# Autodesk Inventor assembly: カート
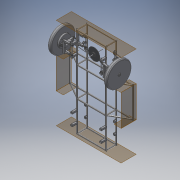
[picture p0: Inventor's stored thumbnail of the model, 180x180]
Saved by Autodesk Inventor 2018 (Build 220112000, 112)
## iProperties
Created: 2017-10-07
Part Number: カート
Material: 一般
Document SubType Name: Assembly
Designer: Kosei
Author: Kosei
## Documents named in this file (17)
- C:\Users\mura5\Documents\RBBR\CAD\カート.iam
- C:\Users\mura5\Documents\RBBR\CAD\シャーシ\シャーシ.iam
- C:\Users\mura5\Documents\RBBR\CAD\サスペンション\上アーム(前).iam
- C:\Users\mura5\Documents\RBBR\CAD\汎用部品\シャフト12x300mm.ipt
- C:\Users\mura5\Documents\RBBR\CAD\サスペンション\下アーム(前後).iam
- C:\Users\mura5\Documents\RBBR\CAD\サスペンション\車軸受け(前,左).iam
- C:\Users\mura5\Documents\RBBR\CAD\汎用部品\シャフト10x230mm.ipt
- C:\Users\mura5\Documents\RBBR\CAD\サスペンション\スプリング\スプリング.iam
- C:\Users\mura5\Documents\RBBR\CAD\車輪\前輪.ipt
- C:\Users\mura5\Documents\RBBR\CAD\車輪\前輪シャフト.ipt
- C:\Users\mura5\Documents\RBBR\CAD\車輪\前輪シャフトワッシャー.ipt
- C:\Users\mura5\Documents\RBBR\CAD\サスペンション\車軸受け(前,右).iam
- C:\Users\mura5\Documents\RBBR\CAD\ステアリング\ロッド.iam
- C:\Users\mura5\Documents\RBBR\CAD\ステアリング\車輪側スプロケット.ipt
- C:\Users\mura5\Documents\RBBR\CAD\装飾(仮)\前後.ipt
- C:\Users\mura5\Documents\RBBR\CAD\装飾(仮)\左右.ipt
- C:\Users\mura5\Documents\RBBR\CAD\装飾(仮)\泥除け1.ipt
## Components (33 placed, 16 different names)
1. シャーシ:1 [sub-assembly] — フラッシュ:2, フラッシュ:3, フラッシュ:4, 円柱状:1, フラッシュ:5, 円柱状:2, フラッシュ:6, 円柱状:3, フラッシュ:7, 円柱状:4, フラッシュ:8, メイト:1, メイト:2, メイト:3, メイト:4, フラッシュ:9, フラッシュ:10, メイト:5, フラッシュ:11, メイト:6, フラッシュ:12, 角度:3, メイト:7, フラッシュ:13, フラッシュ:14, メイト:8, フラッシュ:15, フラッシュ:16, メイト:9, フラッシュ:17, フラッシュ:18, メイト:10, フラッシュ:19, メイト:11, メイト:12, フラッシュ:25, メイト:15, メイト:17
2. 泥除け1:1 — メイト:11, フラッシュ:24, メイト:13
3. 泥除け1:2 — メイト:15, フラッシュ:26, メイト:16
4. 泥除け1:3 — メイト:12, フラッシュ:23, メイト:14
5. 泥除け1:4 — メイト:17, フラッシュ:27, メイト:18
6. シャフト12x300mm:1 — 円柱状:1, フラッシュ:5, 円柱状:5, 円柱状:11
7. シャフト12x300mm:3 — 円柱状:3, フラッシュ:7, 円柱状:7
8. シャフト10x230mm:1 — 円柱状:9, フラッシュ:9, 円柱状:12
9. 上アーム(前):1 [sub-assembly] — 円柱状:5, メイト:1, リジッド:1, 角度:4
10. 下アーム(前後):1 [sub-assembly] — 円柱状:7, メイト:3, リジッド:2, 円柱状:9
11. 車軸受け(前,左):1 [sub-assembly] — リジッド:1, リジッド:2, 回転:2, リジッド:9
12. スプリング:1 [sub-assembly] — 円柱状:11, 円柱状:12
13. 前輪:1 — 回転:1, リジッド:5, 角度:8
14. 前輪シャフト:1 — 回転:1
15. 前輪シャフトワッシャー:1 — リジッド:5, 回転:2
16. シャフト12x300mm:2 — 円柱状:2, フラッシュ:6, 円柱状:6, 円柱状:13
17. シャフト12x300mm:4 — 円柱状:4, フラッシュ:8, 円柱状:8
18. シャフト10x230mm:2 — フラッシュ:10, 円柱状:10, 円柱状:14
19. 上アーム(前):2 [sub-assembly] — 円柱状:6, メイト:2, リジッド:3, 角度:5
20. 下アーム(前後):2 [sub-assembly] — 円柱状:8, メイト:4, リジッド:4, 円柱状:10
21. 車軸受け(前,右):1 [sub-assembly] — リジッド:3, リジッド:4, 回転:3, リジッド:8
22. スプリング:2 [sub-assembly] — 円柱状:13, 円柱状:14
23. 前輪:2 — リジッド:6, リジッド:7
24. 前輪シャフト:2 — リジッド:6
25. 前輪シャフトワッシャー:2 — リジッド:7, 回転:3
26. ロッド:1 [sub-assembly] — リジッド:8, リジッド:12, 角度:6
27. ロッド:2 [sub-assembly] — リジッド:9, リジッド:13, 角度:7
28. 車輪側スプロケット:1 — 円柱状:15, フラッシュ:12, リジッド:12, リジッド:13, 角度:3, 角度:6, 角度:7
29. シャフト12x300mm:5 — メイト:5, フラッシュ:11, メイト:6, 円柱状:15
30. 前後:1 — メイト:7, フラッシュ:13, フラッシュ:14
31. 前後:2 — メイト:8, フラッシュ:15, フラッシュ:16
32. 左右:1 — メイト:9, フラッシュ:17, フラッシュ:18, フラッシュ:26, メイト:16, フラッシュ:27, メイト:18
33. 左右:2 — メイト:10, フラッシュ:19, 角度:8, フラッシュ:23, フラッシュ:24, フラッシュ:25, メイト:13, メイト:14
## Relationships (76: Flush 23, Mate 18, CylindricalJoint 15, WeldJoint 11, Angle 6, RevoluteJoint 3)
- フラッシュ:2 [Flush]: シャーシ:1
- フラッシュ:3 [Flush]: シャーシ:1
- フラッシュ:4 [Flush]: シャーシ:1
- 円柱状:1 [CylindricalJoint]: シャーシ:1 ↔ シャフト12x300mm:1
- フラッシュ:5 [Flush]: シャーシ:1 ↔ シャフト12x300mm:1
- 円柱状:2 [CylindricalJoint]: シャーシ:1 ↔ シャフト12x300mm:2
- フラッシュ:6 [Flush]: シャーシ:1 ↔ シャフト12x300mm:2
- 円柱状:3 [CylindricalJoint]: シャーシ:1 ↔ シャフト12x300mm:3
- フラッシュ:7 [Flush]: シャーシ:1 ↔ シャフト12x300mm:3
- 円柱状:4 [CylindricalJoint]: シャーシ:1 ↔ シャフト12x300mm:4
- フラッシュ:8 [Flush]: シャーシ:1 ↔ シャフト12x300mm:4
- 円柱状:5 [CylindricalJoint]: シャフト12x300mm:1 ↔ 上アーム(前):1
- メイト:1 [Mate]: シャーシ:1 ↔ 上アーム(前):1
- 円柱状:6 [CylindricalJoint]: シャフト12x300mm:2 ↔ 上アーム(前):2
- メイト:2 [Mate]: シャーシ:1 ↔ 上アーム(前):2
- 円柱状:7 [CylindricalJoint]: シャフト12x300mm:3 ↔ 下アーム(前後):1
- メイト:3 [Mate]: シャーシ:1 ↔ 下アーム(前後):1
- 円柱状:8 [CylindricalJoint]: シャフト12x300mm:4 ↔ 下アーム(前後):2
- メイト:4 [Mate]: シャーシ:1 ↔ 下アーム(前後):2
- リジッド:1 [WeldJoint]: 上アーム(前):1 ↔ 車軸受け(前,左):1
- リジッド:2 [WeldJoint]: 下アーム(前後):1 ↔ 車軸受け(前,左):1
- リジッド:3 [WeldJoint]: 上アーム(前):2 ↔ 車軸受け(前,右):1
- リジッド:4 [WeldJoint]: 下アーム(前後):2 ↔ 車軸受け(前,右):1
- 円柱状:9 [CylindricalJoint]: シャフト10x230mm:1 ↔ 下アーム(前後):1
- フラッシュ:9 [Flush]: シャーシ:1 ↔ シャフト10x230mm:1
- フラッシュ:10 [Flush]: シャーシ:1 ↔ シャフト10x230mm:2
- 円柱状:10 [CylindricalJoint]: シャフト10x230mm:2 ↔ 下アーム(前後):2
- 円柱状:11 [CylindricalJoint]: シャフト12x300mm:1 ↔ スプリング:1
- 円柱状:12 [CylindricalJoint]: シャフト10x230mm:1 ↔ スプリング:1
- 円柱状:13 [CylindricalJoint]: シャフト12x300mm:2 ↔ スプリング:2
- 円柱状:14 [CylindricalJoint]: シャフト10x230mm:2 ↔ スプリング:2
- 回転:1 [RevoluteJoint]: 前輪:1 ↔ 前輪シャフト:1
- リジッド:5 [WeldJoint]: 前輪:1 ↔ 前輪シャフトワッシャー:1
- 回転:2 [RevoluteJoint]: 車軸受け(前,左):1 ↔ 前輪シャフトワッシャー:1
- リジッド:6 [WeldJoint]: 前輪:2 ↔ 前輪シャフト:2
- リジッド:7 [WeldJoint]: 前輪:2 ↔ 前輪シャフトワッシャー:2
- 回転:3 [RevoluteJoint]: 車軸受け(前,右):1 ↔ 前輪シャフトワッシャー:2
- リジッド:8 [WeldJoint]: 車軸受け(前,右):1 ↔ ロッド:1
- リジッド:9 [WeldJoint]: 車軸受け(前,左):1 ↔ ロッド:2
- メイト:5 [Mate]: シャーシ:1 ↔ シャフト12x300mm:5
- フラッシュ:11 [Flush]: シャーシ:1 ↔ シャフト12x300mm:5
- メイト:6 [Mate]: シャーシ:1 ↔ シャフト12x300mm:5
- 円柱状:15 [CylindricalJoint]: 車輪側スプロケット:1 ↔ シャフト12x300mm:5
- フラッシュ:12 [Flush] (160 mm): シャーシ:1 ↔ 車輪側スプロケット:1
- リジッド:12 [WeldJoint]: ロッド:1 ↔ 車輪側スプロケット:1
- リジッド:13 [WeldJoint]: ロッド:2 ↔ 車輪側スプロケット:1
- 角度:3 [Angle] (0 deg): シャーシ:1 ↔ 車輪側スプロケット:1
- 角度:4 [Angle] (0 deg): 上アーム(前):1
- 角度:5 [Angle] (10 deg): 上アーム(前):2
- 角度:6 [Angle] (0 deg): ロッド:1 ↔ 車輪側スプロケット:1
- 角度:7 [Angle] (0 deg): ロッド:2 ↔ 車輪側スプロケット:1
- メイト:7 [Mate]: シャーシ:1 ↔ 前後:1
- フラッシュ:13 [Flush] (30 mm): シャーシ:1 ↔ 前後:1
- フラッシュ:14 [Flush] (640 mm): シャーシ:1 ↔ 前後:1
- メイト:8 [Mate]: シャーシ:1 ↔ 前後:2
- フラッシュ:15 [Flush] (30 mm): シャーシ:1 ↔ 前後:2
- フラッシュ:16 [Flush] (640 mm): シャーシ:1 ↔ 前後:2
- メイト:9 [Mate]: シャーシ:1 ↔ 左右:1
- フラッシュ:17 [Flush] (30 mm): シャーシ:1 ↔ 左右:1
- フラッシュ:18 [Flush] (4 mm): シャーシ:1 ↔ 左右:1
- メイト:10 [Mate]: シャーシ:1 ↔ 左右:2
- フラッシュ:19 [Flush] (30 mm): シャーシ:1 ↔ 左右:2
- 角度:8 [Angle] (0 deg): 前輪:1 ↔ 左右:2
- メイト:11 [Mate]: シャーシ:1 ↔ 泥除け1:1
- メイト:12 [Mate]: シャーシ:1 ↔ 泥除け1:3
- フラッシュ:23 [Flush]: 泥除け1:3 ↔ 左右:2
- フラッシュ:24 [Flush]: 泥除け1:1 ↔ 左右:2
- フラッシュ:25 [Flush] (4 mm): シャーシ:1 ↔ 左右:2
- メイト:13 [Mate]: 泥除け1:1 ↔ 左右:2
- メイト:14 [Mate]: 泥除け1:3 ↔ 左右:2
- メイト:15 [Mate]: シャーシ:1 ↔ 泥除け1:2
- フラッシュ:26 [Flush]: 泥除け1:2 ↔ 左右:1
- メイト:16 [Mate]: 泥除け1:2 ↔ 左右:1
- メイト:17 [Mate]: シャーシ:1 ↔ 泥除け1:4
- フラッシュ:27 [Flush]: 泥除け1:4 ↔ 左右:1
- メイト:18 [Mate]: 泥除け1:4 ↔ 左右:1
